# Autodesk Inventor assembly: PCB Component
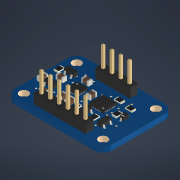
[picture p0: Inventor's stored thumbnail of the model, 180x180]
Saved by Autodesk Inventor 2021 (Build 250183000, 183)
## iProperties
Created: 2021-01-19
Part Number: PCB Component
Document SubType Name: Assembly
Designer: User
Author: User
## Documents named in this file (10)
- D:\SynologyDrive\tcodev\tco-cad\common\adafruit_9dof\adafruit_9dof.iam
- D:\SynologyDrive\tcodev\tco-cad\common\adafruit_9dof\Board.ipt
- D:\SynologyDrive\tcodev\tco-cad\common\kicad_packages_3d\R_0805_2012Metric.ipt
- D:\SynologyDrive\tcodev\tco-cad\common\kicad_packages_3d\C_0805_2012Metric.ipt
- D:\SynologyDrive\tcodev\tco-cad\common\kicad_packages_3d\QFN-16-1EP_3x3mm_P0.5mm_EP1.8x1.8mm.ipt
- D:\SynologyDrive\tcodev\tco-cad\common\kicad_packages_3d\QFN-24-1EP_4x4mm_P0.5mm_EP2.6x2.6mm.ipt
- D:\SynologyDrive\tcodev\tco-cad\common\kicad_packages_3d\SOT-23.ipt
- D:\SynologyDrive\tcodev\tco-cad\common\kicad_packages_3d\D_SOD-323.ipt
- D:\SynologyDrive\tcodev\tco-cad\common\kicad_packages_3d\PinHeader_1x04_P2.54mm_Vertical.ipt
- D:\SynologyDrive\tcodev\tco-cad\common\kicad_packages_3d\PinHeader_1x06_P2.54mm_Vertical.ipt
## Components (23 placed, 9 different names)
1. Board:1 — Mate:1, Mate:2, Rotational:1, Rotational:2
2. R_0805_2012Metric:1
3. C_0805_2012Metric:1
4. C_0805_2012Metric:2
5. C_0805_2012Metric:3
6. C_0805_2012Metric:4
7. C_0805_2012Metric:5
8. R_0805_2012Metric:2
9. R_0805_2012Metric:3
10. R_0805_2012Metric:4
11. R_0805_2012Metric:5
12. C_0805_2012Metric:6
13. C_0805_2012Metric:7
14. R_0805_2012Metric:6
15. QFN-16-1EP_3x3mm_P0.5mm_EP1.8x1.8mm:1
16. QFN-24-1EP_4x4mm_P0.5mm_EP2.6x2.6mm:1
17. SOT-23:1
18. SOT-23:2
19. SOT-23:3
20. SOT-23:4
21. D_SOD-323:1
22. PinHeader_1x06_P2.54mm_Vertical:1 — Mate:2, Rotational:1
23. PinHeader_1x04_P2.54mm_Vertical:1 — Mate:1, Rotational:2
## Relationships (4: Mate 2, RevoluteJoint 2)
- Mate:1: Board:1 ↔ PinHeader_1x04_P2.54mm_Vertical:1
- Mate:2: Board:1 ↔ PinHeader_1x06_P2.54mm_Vertical:1
- Rotational:1 [RevoluteJoint] (-3 mm): Board:1 ↔ PinHeader_1x06_P2.54mm_Vertical:1
- Rotational:2 [RevoluteJoint] (-3 mm): Board:1 ↔ PinHeader_1x04_P2.54mm_Vertical:1
